# Autodesk Inventor assembly: Rotor_assembly
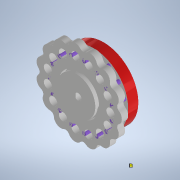
[picture p0: Inventor's stored thumbnail of the model, 180x180]
Saved by Autodesk Inventor 2021 (Build 250183000, 183)
## iProperties
Created: 2022-08-08
Part Number: Rotor_assembly
Document SubType Name: Assembly
Designer: MicnedSQ
Author: MicnedSQ
## Documents named in this file (5)
- C:\Users\MicnedSQ\Desktop\V1\Rotor_assembly.iam
- C:\Users\MicnedSQ\Desktop\V1\Rotor_shaft_2.ipt
- C:\Users\MicnedSQ\Desktop\V1\Rotor_shaft_2_2.ipt
- C:\Users\MicnedSQ\Desktop\V1\Rotor.ipt
- C:\Users\MicnedSQ\Desktop\V1\Część1.ipt
## Components (4 placed, 4 different names)
1. Rotor_shaft_2:1 — Sztywne:1, Obrotowe:1
2. Rotor_shaft_2_2:1 — Sztywne:1, Obrotowe:2
3. Rotor:1 — Obrotowe:1
4. Część1:1 — Obrotowe:2
## Relationships (3: RevoluteJoint 2, WeldJoint 1)
- Sztywne:1 [WeldJoint]: Rotor_shaft_2:1 ↔ Rotor_shaft_2_2:1
- Obrotowe:1 [RevoluteJoint]: Rotor_shaft_2:1 ↔ Rotor:1
- Obrotowe:2 [RevoluteJoint]: Rotor_shaft_2_2:1 ↔ Część1:1
